# Autodesk Inventor assembly: КВ33.044.700 - Шкив плоский Makeblock сборка
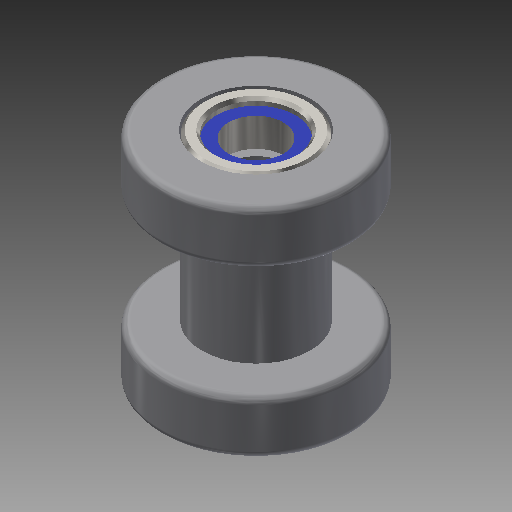
[picture p0: Inventor's stored thumbnail of the model, 512x512]
Saved by Autodesk Inventor 2019 (Build 230136000, 136)
## iProperties
Created: 2019-08-06
Part Number: КВ33.044.700 - Шкив плоский Makeblock сборка
Material: Типовые
Document SubType Name: Assembly
Designer: Петров Иван
Author: Петров Иван
## Documents named in this file (3)
- E:\IVAN\Kvantoriada2019\optimal_gripper\hardware\Стандартные изделия\Шкив плоский Makeblock сборка.iam
- E:\IVAN\Kvantoriada2019\optimal_gripper\hardware\Стандартные изделия\Подшипник 4x8x3.ipt
- E:\IVAN\Kvantoriada2019\optimal_gripper\hardware\Стандартные изделия\Шкив плоский Makeblock.ipt
## Components (3 placed, 2 different names)
1. Подшипник 4x8x3:1 — Совмещение:3, Совмещение:4
2. Подшипник 4x8x3:2 — Совмещение:1, Совмещение:2
3. Шкив плоский Makeblock:1 — Совмещение:1, Совмещение:2, Совмещение:3, Совмещение:4
## Relationships (4: Mate 4)
- Совмещение:1 [Mate]: Подшипник 4x8x3:2 ↔ Шкив плоский Makeblock:1
- Совмещение:2 [Mate]: Подшипник 4x8x3:2 ↔ Шкив плоский Makeblock:1
- Совмещение:3 [Mate]: Подшипник 4x8x3:1 ↔ Шкив плоский Makeblock:1
- Совмещение:4 [Mate]: Подшипник 4x8x3:1 ↔ Шкив плоский Makeblock:1
